# Autodesk Inventor assembly: 組合檔
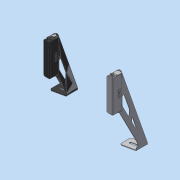
[picture p0: Inventor's stored thumbnail of the model, 180x180]
Saved by Autodesk Inventor 2020 (Build 240168000, 168)
## iProperties
Created: 2015-11-28
Part Number: 組合檔
Document SubType Name: Assembly
Designer: 設計製圖
Author: 設計製圖
## Documents named in this file (5)
- D:\資料庫\設計-3D產品\【May club 】\得利卡-車頂燈架\模型、圖面\差異比較-黑鐵、白鐵.iam
- D:\資料庫\設計-3D產品\【May club 】\得利卡-車頂燈架\模型、圖面\車頂燈架長-組合(白鐵).iam
- D:\資料庫\設計-3D產品\【May club 】\得利卡-車頂燈架\模型、圖面\黑鐵版本\車頂燈架長-組合(黑鐵).iam
- D:\資料庫\設計-3D產品\【May club 】\得利卡-車頂燈架\模型、圖面\車頂燈架短-組合(白鐵).iam
- D:\資料庫\設計-3D產品\【May club 】\得利卡-車頂燈架\模型、圖面\黑鐵版本\車頂燈架短-組合(黑鐵).iam
## Components (4 placed, 4 different names)
1. 車頂燈架長-組合(白鐵):1 [sub-assembly] — 齊平:1, 齊平:2, 齊平:3, 齊平:4, 齊平:5
2. 車頂燈架長-組合(黑鐵):1 [sub-assembly] — 齊平:1, 齊平:2, 齊平:3
3. 車頂燈架短-組合(白鐵):1 [sub-assembly] — 齊平:4, 齊平:5, 齊平:6, 齊平:7, 齊平:8
4. 車頂燈架短-組合(黑鐵):1 [sub-assembly] — 齊平:6, 齊平:7, 齊平:8
## Relationships (8: Flush 8)
- 齊平:1 [Flush]: 車頂燈架長-組合(白鐵):1 ↔ 車頂燈架長-組合(黑鐵):1
- 齊平:2 [Flush]: 車頂燈架長-組合(白鐵):1 ↔ 車頂燈架長-組合(黑鐵):1
- 齊平:3 [Flush]: 車頂燈架長-組合(白鐵):1 ↔ 車頂燈架長-組合(黑鐵):1
- 齊平:4 [Flush]: 車頂燈架長-組合(白鐵):1 ↔ 車頂燈架短-組合(白鐵):1
- 齊平:5 [Flush]: 車頂燈架長-組合(白鐵):1 ↔ 車頂燈架短-組合(白鐵):1
- 齊平:6 [Flush]: 車頂燈架短-組合(白鐵):1 ↔ 車頂燈架短-組合(黑鐵):1
- 齊平:7 [Flush]: 車頂燈架短-組合(白鐵):1 ↔ 車頂燈架短-組合(黑鐵):1
- 齊平:8 [Flush]: 車頂燈架短-組合(白鐵):1 ↔ 車頂燈架短-組合(黑鐵):1
